# Autodesk Inventor assembly: FullBot
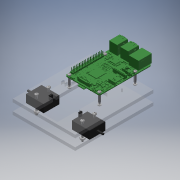
[picture p0: Inventor's stored thumbnail of the model, 180x180]
Saved by Autodesk Inventor 2018 (Build 220112000, 112)
## iProperties
Created: 2018-05-04
Part Number: FullBot
Document SubType Name: Assembly
Designer: mmarkle
Author: mmarkle
## Documents named in this file (9)
- C:\Users\mmarkle\Documents\Robotics\PiBots2018\FullBot.iam
- C:\Users\mmarkle\Documents\Robotics\PiBots2018\pibot_baseplate.ipt
- C:\Users\mmarkle\Documents\Robotics\PiBots2018\MotorWithEnclosure.ipt
- C:\Users\mmarkle\Documents\Robotics\PiBots2018\pibot_baseplate_battery.ipt
- C:\Users\mmarkle\Documents\Robotics\PiBots2018\Raspberry Pi 3_Shrinkwrap_1.ipt
- C:\Users\mmarkle\Documents\Robotics\PiBots2018\FullBot\Design Accelerator\Bolted Connection1.iam
- C:\Users\mmarkle\Documents\Robotics\PiBots2018\12mm_M2.5_standoff.ipt
- C:\Users\mmarkle\Documents\Robotics\PiBots2018\FullBot\Design Accelerator\Bolted Connection2.iam
- C:\Users\mmarkle\Documents\Robotics\PiBots2018\FullBot\Design Accelerator\Bolted Connection3.iam
## Components (12 placed, 8 different names)
1. pibot_baseplate:1 — Mate:1, Mate:2, Mate:3, Mate:4, Mate:5, Mate:6
2. MotorWithEnclosure:1 — Mate:2, Mate:3, Mate:6, Mate:8
3. MotorWithEnclosure:2 — Mate:1, Mate:4, Mate:5, Mate:7, Mate:9
4. pibot_baseplate_battery:1 — Mate:7, Mate:8, Mate:9, Mate:12, Mate:13, Angle:1, Mate:14, Mate:15, Mate:16, Mate:17, Mate:18, Mate:19, Mate:20, Mate:21, Mate:29, Mate:30, Mate:46, Mate:47, Mate:48
5. Raspberry Pi 3:1 — Mate:12, Mate:13, Angle:1, Mate:22, Mate:45
6. MotorScrews [sub-assembly] — Mate:47, Mate:48
7. 12mm_M2.5_standoff:1 — Mate:16, Mate:18
8. 12mm_M2.5_standoff:2 — Mate:14, Mate:21
9. 12mm_M2.5_standoff:3 — Mate:15, Mate:20, Mate:22
10. 12mm_M2.5_standoff:4 — Mate:17, Mate:19
11. TopPiScrews [sub-assembly] — Mate:45, Mate:46
12. BottomPiScrews [sub-assembly] — Mate:29, Mate:30
## Relationships (27: Mate 26, Angle 1)
- Mate:1: pibot_baseplate:1 ↔ MotorWithEnclosure:2
- Mate:2: pibot_baseplate:1 ↔ MotorWithEnclosure:1
- Mate:3: pibot_baseplate:1 ↔ MotorWithEnclosure:1
- Mate:4: pibot_baseplate:1 ↔ MotorWithEnclosure:2
- Mate:5: pibot_baseplate:1 ↔ MotorWithEnclosure:2
- Mate:6: pibot_baseplate:1 ↔ MotorWithEnclosure:1
- Mate:7: MotorWithEnclosure:2 ↔ pibot_baseplate_battery:1
- Mate:8: MotorWithEnclosure:1 ↔ pibot_baseplate_battery:1
- Mate:9: MotorWithEnclosure:2 ↔ pibot_baseplate_battery:1
- Mate:12: pibot_baseplate_battery:1 ↔ Raspberry Pi 3:1
- Mate:13: pibot_baseplate_battery:1 ↔ Raspberry Pi 3:1
- Angle:1 (0 deg): pibot_baseplate_battery:1 ↔ Raspberry Pi 3:1
- Mate:14: pibot_baseplate_battery:1 ↔ 12mm_M2.5_standoff:2
- Mate:15: pibot_baseplate_battery:1 ↔ 12mm_M2.5_standoff:3
- Mate:16: pibot_baseplate_battery:1 ↔ 12mm_M2.5_standoff:1
- Mate:17: pibot_baseplate_battery:1 ↔ 12mm_M2.5_standoff:4
- Mate:18: pibot_baseplate_battery:1 ↔ 12mm_M2.5_standoff:1
- Mate:19: pibot_baseplate_battery:1 ↔ 12mm_M2.5_standoff:4
- Mate:20: pibot_baseplate_battery:1 ↔ 12mm_M2.5_standoff:3
- Mate:21: pibot_baseplate_battery:1 ↔ 12mm_M2.5_standoff:2
- Mate:22: Raspberry Pi 3:1 ↔ 12mm_M2.5_standoff:3
- Mate:29: pibot_baseplate_battery:1 ↔ BottomPiScrews
- Mate:30: pibot_baseplate_battery:1 ↔ BottomPiScrews
- Mate:45: Raspberry Pi 3:1 ↔ TopPiScrews
- Mate:46: pibot_baseplate_battery:1 ↔ TopPiScrews
- Mate:47: pibot_baseplate_battery:1 ↔ MotorScrews
- Mate:48: pibot_baseplate_battery:1 ↔ MotorScrews
